# Autodesk Inventor assembly: Walls
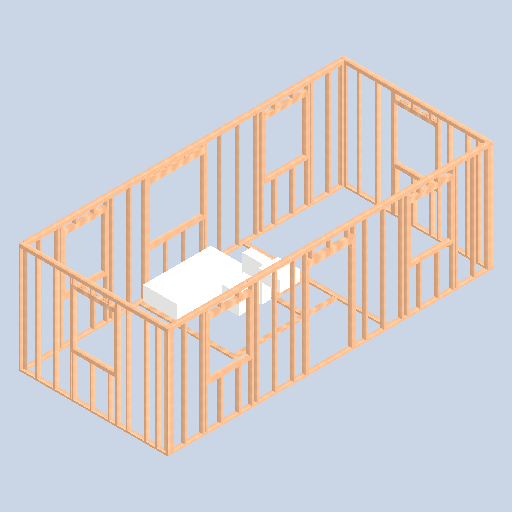
[picture p0: Inventor's stored thumbnail of the model, 512x512]
Saved by Autodesk Inventor 2025 (Build 290162010, 162A)
## iProperties
Created: 2024-09-15
Part Number: Walls
Document SubType Name: Assembly
Designer: Tom
Author: Tom
## Documents named in this file (19)
- C:\Users\Tom\Documents\Inventor\Mobility\Additional_Building\Framing_For_First_Floor.iam
- C:\Users\Tom\Documents\Inventor\Mobility\Additional_Building\Plate_With_Length_144_Inches.ipt
- C:\Users\Tom\Documents\Inventor\Mobility\Additional_Building\Plate_With_Length_125_Inches.ipt
- C:\Users\Tom\Documents\Inventor\Mobility\Additional_Building\California_Corner.iam
- C:\Users\Tom\Documents\Inventor\Mobility\Additional_Building\Stud_With_Height_93_Inches.ipt
- C:\Users\Tom\Documents\Inventor\Mobility\Additional_Building\Plate_With_Length_132_Inches.ipt
- C:\Users\Tom\Documents\Inventor\Mobility\Additional_Building\Plate_With_Length_68.5_Inches.ipt
- C:\Users\Tom\Documents\Inventor\Mobility\Additional_Building\Plate_With_Length_83.350_Inches.ipt
- C:\Users\Tom\Documents\Inventor\Mobility\Additional_Building\Plate_With_Length_60_Inches.ipt
- C:\Users\Tom\Documents\Inventor\Mobility\Additional_Building\Plate_With_Length_25_Inches.ipt
- C:\Users\Tom\Documents\Inventor\Mobility\Additional_Building\Stud_With_Height_80.5_Inches.ipt
- C:\Users\Tom\Documents\Inventor\Mobility\Additional_Building\Stud_With_Height_7_Inches.ipt
- C:\Users\Tom\Documents\Inventor\Mobility\Additional_Building\Framing_For_First_Floor_Window.iam
- C:\Users\Tom\Documents\Inventor\Mobility\Additional_Building\Framing_For_Side_Window.iam
- C:\Users\Tom\Documents\Inventor\Mobility\Additional_Building\Framing_For_Bathroom_Window.iam
- C:\Users\Tom\Documents\Inventor\Mobility\Bathtub.ipt
- C:\Users\Tom\Documents\Inventor\Mobility\Toilet.ipt
- C:\Users\Tom\Documents\Inventor\Mobility\Bathroom_Sink.ipt
- C:\Users\Tom\Documents\Inventor\Mobility\Additional_Building\Header_With_Dimensions_3.5_x_5.5_x_41.25_Inches.iam
## Components (78 placed, 18 different names)
1. California_Corner:1 [sub-assembly] — Mate:2, Flush:3, Flush:4, Flush:95
2. California_Corner:2 [sub-assembly] — Mate:13, Flush:13, Flush:14, Flush:19, Flush:20, Flush:31, Mate:34, Flush:64, Flush:70
3. California_Corner:3 [sub-assembly] — Mate:14, Flush:15, Flush:16
4. California_Corner:4 [sub-assembly] — Mate:15, Flush:17, Flush:18
5. Plate_With_Length_125_Inches:5 — Mate:16, Flush:22, Mate:17, Mate:24
6. Plate_With_Length_60_Inches:1 — Mate:27, Flush:44, Flush:101, Flush:102, Mate:95
7. Plate_With_Length_25_Inches:1 — Mate:25, Mate:28, Flush:103
8. Plate_With_Length_25_Inches:2 — Mate:24, Mate:25, Mate:29
9. Plate_With_Length_83.350_Inches:1 — Mate:26, Mate:27, Mate:28, Mate:29, Flush:44, Mate:91, Flush:100, Mate:92, Mate:94, Flush:103
10. Plate_With_Length_83.350_Inches:2 — Mate:30, Mate:79, Flush:102, Mate:95
11. Stud_With_Height_93_Inches:56 — Mate:33, Flush:32, Mate:34, Mate:39, Mate:101, Flush:108
12. Stud_With_Height_93_Inches:57 — Mate:36, Flush:35, Mate:41
13. Stud_With_Height_80.5_Inches:1 — Mate:38, Flush:36, Mate:39, Mate:100
14. Stud_With_Height_80.5_Inches:2 — Mate:40, Flush:37, Mate:41
15. Framing_For_Bathroom_Window:1 [sub-assembly] — Mate:78, Flush:86, Mate:79, Mate:98
16. Bathtub:1 — Mate:90, Mate:91, Mate:93
17. Toilet:1 — Flush:100, Mate:92, Mate:93
18. Bathroom_Sink:1 — Mate:94, Flush:101
19. Stud_With_Height_93_Inches:103 — Mate:97, Flush:106, Mate:98
20. Header_With_Dimensions_3.5_x_5.5_x_41.25_Inches:1 [sub-assembly] — Mate:100, Mate:101, Flush:108
21. Plate_With_Length_132_Inches:1 — Mate:8, Flush:9, Flush:10, Mate:10
22. Plate_With_Length_132_Inches:2
23. Plate_With_Length_144_Inches:9 — Mate:11, Mate:12, Flush:12
24. Plate_With_Length_144_Inches:10
25. Stud_With_Height_7_Inches:1 — Flush:39, Mate:99, Flush:107
26. Stud_With_Height_7_Inches:2
27. Stud_With_Height_7_Inches:3
28. Stud_With_Height_93_Inches:49 — Mate:32, Flush:30, Flush:31
29. Framing_For_Side_Window:1 [sub-assembly] — Mate:65, Flush:69, Flush:70
30. Stud_With_Height_93_Inches:71
31. Framing_For_Side_Window:2 [sub-assembly]
32. Stud_With_Height_93_Inches:62 — Mate:61, Flush:61, Flush:88
33. Stud_With_Height_93_Inches:63
34. Stud_With_Height_93_Inches:85
35. Framing_For_First_Floor_Window:1 [sub-assembly] — Mate:62, Flush:63, Flush:64
36. Framing_For_First_Floor_Window:2 [sub-assembly] — Flush:94, Mate:86, Flush:95, Flush:98
37. Framing_For_First_Floor_Window:3 [sub-assembly] — Flush:105
38. Framing_For_First_Floor_Window:4 [sub-assembly]
39. Stud_With_Height_93_Inches:101 — Mate:96, Flush:104, Flush:105
40. Stud_With_Height_93_Inches:102
41. Plate_With_Length_144_Inches:1 — Flush:5, Mate:15, Flush:17, Flush:18, Mate:30, Mate:78, Flush:86, Mate:96, Flush:104, Mate:97, Flush:106
42. Plate_With_Length_144_Inches:2 — Mate:14, Flush:15, Flush:16, Mate:26, Mate:90
43. Plate_With_Length_144_Inches:3 — Mate:1, Flush:1, Flush:2, Mate:4, Flush:6, Mate:13, Flush:13, Flush:14, Mate:16, Flush:22, Mate:33, Flush:32, Mate:38, Flush:36, Mate:61, Flush:61, Mate:62, Flush:63
44. Plate_With_Length_144_Inches:4 — Mate:2, Flush:3, Flush:4, Mate:36, Flush:35, Mate:40, Flush:37, Mate:44, Flush:42, Flush:94, Mate:86, Mate:89, Flush:97
45. Plate_With_Length_125_Inches:1 — Mate:1, Flush:1, Flush:2, Mate:3, Mate:7, Mate:32, Flush:30, Mate:65, Flush:69, Mate:66, Flush:71
46. Plate_With_Length_125_Inches:2 — Mate:17
47. Plate_With_Length_144_Inches:5 — Flush:9
48. Plate_With_Length_144_Inches:6
49. Plate_With_Length_144_Inches:7 — Mate:9, Flush:11, Mate:99, Flush:107
50. Plate_With_Length_144_Inches:8 — Mate:11, Flush:12
51. Plate_With_Length_125_Inches:3 — Flush:7, Mate:8, Flush:10
52. Plate_With_Length_125_Inches:4
53. Plate_With_Length_68.5_Inches:1 — Mate:9, Mate:10, Flush:11
54. Plate_With_Length_68.5_Inches:2 — Mate:12
55. Plate_With_Length_68.5_Inches:3
56. Plate_With_Length_68.5_Inches:4
57. Stud_With_Height_93_Inches:23 — Flush:7, Mate:7, Flush:20, Flush:72
58. Stud_With_Height_93_Inches:68
59. Stud_With_Height_93_Inches:69 — Mate:66, Flush:71, Flush:72
60. Stud_With_Height_93_Inches:70
61. Stud_With_Height_93_Inches:72
62. Stud_With_Height_93_Inches:73
63. Stud_With_Height_93_Inches:74
64. Stud_With_Height_93_Inches:75
65. Stud_With_Height_93_Inches:1 — Mate:4, Flush:6, Flush:19, Flush:39, Flush:43, Flush:88
66. Stud_With_Height_93_Inches:92
67. Stud_With_Height_93_Inches:58 — Mate:44, Flush:42, Flush:43
68. Stud_With_Height_93_Inches:64
69. Stud_With_Height_93_Inches:86
70. Stud_With_Height_93_Inches:91 — Mate:89, Flush:97, Flush:98
71. Stud_With_Height_93_Inches:93
72. Stud_With_Height_93_Inches:94
73. Stud_With_Height_93_Inches:95
74. Stud_With_Height_93_Inches:96
75. Stud_With_Height_93_Inches:97
76. Stud_With_Height_93_Inches:98
77. Stud_With_Height_93_Inches:99
78. Stud_With_Height_93_Inches:100
## Component patterns: (2 elements), (2 elements, first: Plate_With_Length_132_Inches:1), (2 elements, first: Plate_With_Length_144_Inches:9), (3 elements, first: Stud_With_Height_7_Inches:1), (2 elements, first: Stud_With_Height_93_Inches:49 + Framing_For_Side_Window:1), (3 elements, first: Stud_With_Height_93_Inches:62), (2 elements, first: Framing_For_First_Floor_Window:1 + Framing_For_First_Floor_Window:2), (2 elements, first: Stud_With_Height_93_Inches:101), (4 elements, first: Plate_With_Length_144_Inches:1), (2 elements, first: Plate_With_Length_125_Inches:1), Component Pattern 1:2 (4 elements), Component Pattern 2:2 (2 elements), (2 elements, first: Plate_With_Length_68.5_Inches:1), Component Pattern 10:2 (2 elements), (2 elements, first: Stud_With_Height_93_Inches:23), (2 elements, first: Stud_With_Height_93_Inches:69), Component Pattern 22:2 (2 elements), Component Pattern 23:2 (2 elements), (2 elements, first: Stud_With_Height_93_Inches:1), (3 elements, first: Stud_With_Height_93_Inches:58), (2 elements, first: Stud_With_Height_93_Inches:91), Component Pattern 31:2 (2 elements), Component Pattern 20:2 (3 elements), Component Pattern 32:2 (2 elements)
## Relationships (103: Flush 52, Mate 51)
- Mate:1: Plate_With_Length_144_Inches:3 ↔ Plate_With_Length_125_Inches:1
- Flush:1: Plate_With_Length_144_Inches:3 ↔ Plate_With_Length_125_Inches:1
- Flush:2: Plate_With_Length_144_Inches:3 ↔ Plate_With_Length_125_Inches:1
- Mate:2: California_Corner:1 ↔ Plate_With_Length_144_Inches:4
- Flush:3: California_Corner:1 ↔ Plate_With_Length_144_Inches:4
- Flush:4: California_Corner:1 ↔ Plate_With_Length_144_Inches:4
- Flush:5: Plate_With_Length_144_Inches:1
- Mate:3 (1536.7 mm): Plate_With_Length_125_Inches:1
- Mate:4: Plate_With_Length_144_Inches:3 ↔ Stud_With_Height_93_Inches:1
- Flush:6: Plate_With_Length_144_Inches:3 ↔ Stud_With_Height_93_Inches:1
- Flush:7: Plate_With_Length_125_Inches:3 ↔ Stud_With_Height_93_Inches:23
- Mate:7: Plate_With_Length_125_Inches:1 ↔ Stud_With_Height_93_Inches:23
- Mate:8: Plate_With_Length_132_Inches:1 ↔ Plate_With_Length_125_Inches:3
- Flush:9: Plate_With_Length_132_Inches:1 ↔ Plate_With_Length_144_Inches:5
- Flush:10: Plate_With_Length_132_Inches:1 ↔ Plate_With_Length_125_Inches:3
- Mate:9: Plate_With_Length_144_Inches:7 ↔ Plate_With_Length_68.5_Inches:1
- Mate:10: Plate_With_Length_132_Inches:1 ↔ Plate_With_Length_68.5_Inches:1
- Flush:11: Plate_With_Length_144_Inches:7 ↔ Plate_With_Length_68.5_Inches:1
- Mate:11: Plate_With_Length_144_Inches:9 ↔ Plate_With_Length_144_Inches:8
- Mate:12: Plate_With_Length_144_Inches:9 ↔ Plate_With_Length_68.5_Inches:2
- Flush:12: Plate_With_Length_144_Inches:9 ↔ Plate_With_Length_144_Inches:8
- Mate:13: California_Corner:2 ↔ Plate_With_Length_144_Inches:3
- Flush:13: California_Corner:2 ↔ Plate_With_Length_144_Inches:3
- Flush:14: California_Corner:2 ↔ Plate_With_Length_144_Inches:3
- Mate:14: California_Corner:3 ↔ Plate_With_Length_144_Inches:2
- Flush:15: California_Corner:3 ↔ Plate_With_Length_144_Inches:2
- Flush:16: California_Corner:3 ↔ Plate_With_Length_144_Inches:2
- Mate:15: California_Corner:4 ↔ Plate_With_Length_144_Inches:1
- Flush:17: California_Corner:4 ↔ Plate_With_Length_144_Inches:1
- Flush:18: California_Corner:4 ↔ Plate_With_Length_144_Inches:1
- Flush:19 (387.35 mm): California_Corner:2 ↔ Stud_With_Height_93_Inches:1
- Flush:20 (501.65 mm): California_Corner:2 ↔ Stud_With_Height_93_Inches:23
- Mate:16: Plate_With_Length_125_Inches:5 ↔ Plate_With_Length_144_Inches:3
- Flush:22: Plate_With_Length_125_Inches:5 ↔ Plate_With_Length_144_Inches:3
- Mate:17 (2184.4 mm): Plate_With_Length_125_Inches:5 ↔ Plate_With_Length_125_Inches:2
- Mate:24: Plate_With_Length_125_Inches:5 ↔ Plate_With_Length_25_Inches:2
- Mate:25 (635 mm): Plate_With_Length_25_Inches:1 ↔ Plate_With_Length_25_Inches:2
- Mate:26: Plate_With_Length_83.350_Inches:1 ↔ Plate_With_Length_144_Inches:2
- Mate:27: Plate_With_Length_60_Inches:1 ↔ Plate_With_Length_83.350_Inches:1
- Mate:28: Plate_With_Length_25_Inches:1 ↔ Plate_With_Length_83.350_Inches:1
- Mate:29: Plate_With_Length_25_Inches:2 ↔ Plate_With_Length_83.350_Inches:1
- Mate:30: Plate_With_Length_83.350_Inches:2 ↔ Plate_With_Length_144_Inches:1
- Mate:32: Stud_With_Height_93_Inches:49 ↔ Plate_With_Length_125_Inches:1
- Flush:30: Stud_With_Height_93_Inches:49 ↔ Plate_With_Length_125_Inches:1
- Flush:31 (250.825 mm): California_Corner:2 ↔ Stud_With_Height_93_Inches:49
- Mate:33: Stud_With_Height_93_Inches:56 ↔ Plate_With_Length_144_Inches:3
- Flush:32: Stud_With_Height_93_Inches:56 ↔ Plate_With_Length_144_Inches:3
- Mate:34 (-3133.725 mm): California_Corner:2 ↔ Stud_With_Height_93_Inches:56
- Mate:36: Stud_With_Height_93_Inches:57 ↔ Plate_With_Length_144_Inches:4
- Flush:35: Stud_With_Height_93_Inches:57 ↔ Plate_With_Length_144_Inches:4
- Mate:38: Stud_With_Height_80.5_Inches:1 ↔ Plate_With_Length_144_Inches:3
- Flush:36: Stud_With_Height_80.5_Inches:1 ↔ Plate_With_Length_144_Inches:3
- Mate:39: Stud_With_Height_93_Inches:56 ↔ Stud_With_Height_80.5_Inches:1
- Mate:40: Stud_With_Height_80.5_Inches:2 ↔ Plate_With_Length_144_Inches:4
- Flush:37: Stud_With_Height_80.5_Inches:2 ↔ Plate_With_Length_144_Inches:4
- Mate:41: Stud_With_Height_93_Inches:57 ↔ Stud_With_Height_80.5_Inches:2
- Flush:39 (2844.8 mm): Stud_With_Height_7_Inches:1 ↔ Stud_With_Height_93_Inches:1
- Mate:44: Plate_With_Length_144_Inches:4 ↔ Stud_With_Height_93_Inches:58
- Flush:42: Plate_With_Length_144_Inches:4 ↔ Stud_With_Height_93_Inches:58
- Flush:43 (4064 mm): Stud_With_Height_93_Inches:1 ↔ Stud_With_Height_93_Inches:58
- Flush:44: Plate_With_Length_60_Inches:1 ↔ Plate_With_Length_83.350_Inches:1
- Mate:61: Stud_With_Height_93_Inches:62 ↔ Plate_With_Length_144_Inches:3
- Flush:61: Stud_With_Height_93_Inches:62 ↔ Plate_With_Length_144_Inches:3
- Mate:62: Framing_For_First_Floor_Window:1 ↔ Plate_With_Length_144_Inches:3
- Flush:63: Framing_For_First_Floor_Window:1 ↔ Plate_With_Length_144_Inches:3
- Flush:64 (865.1875 mm): California_Corner:2 ↔ Framing_For_First_Floor_Window:1
- Mate:65: Framing_For_Side_Window:1 ↔ Plate_With_Length_125_Inches:1
- Flush:69: Framing_For_Side_Window:1 ↔ Plate_With_Length_125_Inches:1
- Flush:70 (1143 mm): California_Corner:2 ↔ Framing_For_Side_Window:1
- Mate:66: Plate_With_Length_125_Inches:1 ↔ Stud_With_Height_93_Inches:69
- Flush:71: Plate_With_Length_125_Inches:1 ↔ Stud_With_Height_93_Inches:69
- Flush:72 (2032 mm): Stud_With_Height_93_Inches:23 ↔ Stud_With_Height_93_Inches:69
- Mate:78: Framing_For_Bathroom_Window:1 ↔ Plate_With_Length_144_Inches:1
- Flush:86: Framing_For_Bathroom_Window:1 ↔ Plate_With_Length_144_Inches:1
- Mate:79 (85.725 mm): Plate_With_Length_83.350_Inches:2 ↔ Framing_For_Bathroom_Window:1
- Flush:88 (1625.6 mm): Stud_With_Height_93_Inches:62 ↔ Stud_With_Height_93_Inches:1
- Flush:94: Framing_For_First_Floor_Window:2 ↔ Plate_With_Length_144_Inches:4
- Mate:86: Framing_For_First_Floor_Window:2 ↔ Plate_With_Length_144_Inches:4
- Flush:95 (865.1875 mm): California_Corner:1 ↔ Framing_For_First_Floor_Window:2
- Mate:89: Plate_With_Length_144_Inches:4 ↔ Stud_With_Height_93_Inches:91
- Flush:97: Plate_With_Length_144_Inches:4 ↔ Stud_With_Height_93_Inches:91
- Flush:98 (406.4 mm): Framing_For_First_Floor_Window:2 ↔ Stud_With_Height_93_Inches:91
- Mate:90: Bathtub:1 ↔ Plate_With_Length_144_Inches:2
- Mate:91: Plate_With_Length_83.350_Inches:1 ↔ Bathtub:1
- Flush:100: Plate_With_Length_83.350_Inches:1 ↔ Toilet:1
- Mate:92 (12.7 mm): Plate_With_Length_83.350_Inches:1 ↔ Toilet:1
- Mate:93 (160.02 mm): Bathtub:1 ↔ Toilet:1
- Mate:94 (12.7 mm): Plate_With_Length_83.350_Inches:1 ↔ Bathroom_Sink:1
- Flush:101 (669.29 mm): Plate_With_Length_60_Inches:1 ↔ Bathroom_Sink:1
- Flush:102: Plate_With_Length_60_Inches:1 ↔ Plate_With_Length_83.350_Inches:2
- Mate:95: Plate_With_Length_60_Inches:1 ↔ Plate_With_Length_83.350_Inches:2
- Flush:103: Plate_With_Length_25_Inches:1 ↔ Plate_With_Length_83.350_Inches:1
- Mate:96: Stud_With_Height_93_Inches:101 ↔ Plate_With_Length_144_Inches:1
- Flush:104: Stud_With_Height_93_Inches:101 ↔ Plate_With_Length_144_Inches:1
- Flush:105 (406.4 mm): Framing_For_First_Floor_Window:3 ↔ Stud_With_Height_93_Inches:101
- Mate:97: Stud_With_Height_93_Inches:103 ↔ Plate_With_Length_144_Inches:1
- Flush:106: Stud_With_Height_93_Inches:103 ↔ Plate_With_Length_144_Inches:1
- Mate:98: Framing_For_Bathroom_Window:1 ↔ Stud_With_Height_93_Inches:103
- Mate:99: Stud_With_Height_7_Inches:1 ↔ Plate_With_Length_144_Inches:7
- Flush:107: Stud_With_Height_7_Inches:1 ↔ Plate_With_Length_144_Inches:7
- Mate:100: Stud_With_Height_80.5_Inches:1 ↔ Header_With_Dimensions_3.5_x_5.5_x_41.25_Inches:1
- Mate:101: Stud_With_Height_93_Inches:56 ↔ Header_With_Dimensions_3.5_x_5.5_x_41.25_Inches:1
- Flush:108: Stud_With_Height_93_Inches:56 ↔ Header_With_Dimensions_3.5_x_5.5_x_41.25_Inches:1
